# Autodesk Inventor assembly: Top_Rail_Full_Small
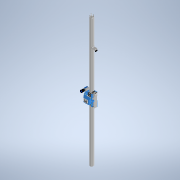
[picture p0: Inventor's stored thumbnail of the model, 180x180]
Saved by Autodesk Inventor 2022 (Build 260153000, 153)
## iProperties
Created: 2022-01-15
Part Number: Top_Rail_Full_Small
Document SubType Name: Assembly
Designer: Jorian Brusind
Description: Top rail assembly for y axis
Author: Jorian Brusind
Revision Number: 2.0
## Documents named in this file (7)
- C:\Users\Jorian Brusind\Documents\GitHub\HyperRail\Inventor Files\Top_Rail_Full_Small.iam
- C:\Users\Jorian Brusind\Documents\GitHub\HyperRail\Inventor Files\Top_Rail_Section.iam
- C:\Users\Jorian Brusind\Documents\GitHub\HyperRail\Inventor Files\MagnetActuatorHolder.ipt
- C:\Users\Jorian Brusind\Documents\GitHub\HyperRail\Inventor Files\59145_Sensor.ipt
- C:\Users\Jorian Brusind\Documents\GitHub\HyperRail\Inventor Files\McMaster Files\Belts\7959K23_1 2 Width MXL Series No. Ll050mxl Timing Belt_20ft.ipt
- C:\Users\Jorian Brusind\Documents\GitHub\HyperRail\Inventor Files\YAxis_Carriage.iam
- C:\Users\Jorian Brusind\Documents\GitHub\HyperRail\Inventor Files\McMaster Files\Belts\7959K23_1 2 Width MXL Series No. Ll050mxl Timing Belt_small.ipt
## Components (6 placed, 6 different names)
1. Top_Rail_Section:1 [sub-assembly] — Flush:6, Mate:26, Mate:27, Mate:28, Flush:14
2. MagnetActuatorHolder:1 — Flush:6, Mate:8, Mate:9, Angle:2
3. 59145_Sensor:2 — Mate:8, Mate:9, Angle:2
4. 7959K23_1 2 Width MXL Series No. Ll050mxl Timing Belt_20ft:1 — Flush:13, Mate:21, Flush:14
5. YAxis_Carriage:1 [sub-assembly] — Mate:22, Mate:26, Mate:27, Mate:28
6. 7959K23_1 2 Width MXL Series No. Ll050mxl Timing Belt_small:1 — Flush:13, Mate:21, Mate:22
## Relationships (11: Mate 7, Flush 3, Angle 1)
- Flush:6 (400 mm): Top_Rail_Section:1 ↔ MagnetActuatorHolder:1
- Mate:8: MagnetActuatorHolder:1 ↔ 59145_Sensor:2
- Mate:9: MagnetActuatorHolder:1 ↔ 59145_Sensor:2
- Angle:2 (0 deg): MagnetActuatorHolder:1 ↔ 59145_Sensor:2
- Flush:13: 7959K23_1 2 Width MXL Series No. Ll050mxl Timing Belt_20ft:1 ↔ 7959K23_1 2 Width MXL Series No. Ll050mxl Timing Belt_small:1
- Mate:21: 7959K23_1 2 Width MXL Series No. Ll050mxl Timing Belt_20ft:1 ↔ 7959K23_1 2 Width MXL Series No. Ll050mxl Timing Belt_small:1
- Mate:22: YAxis_Carriage:1 ↔ 7959K23_1 2 Width MXL Series No. Ll050mxl Timing Belt_small:1
- Mate:26 (12 mm): Top_Rail_Section:1 ↔ YAxis_Carriage:1
- Mate:27 (12 mm): Top_Rail_Section:1 ↔ YAxis_Carriage:1
- Mate:28 (22 mm): Top_Rail_Section:1 ↔ YAxis_Carriage:1
- Flush:14: Top_Rail_Section:1 ↔ 7959K23_1 2 Width MXL Series No. Ll050mxl Timing Belt_20ft:1
